# Autodesk Inventor assembly: Сборка1
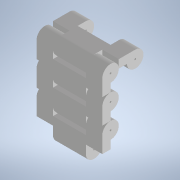
[picture p0: Inventor's stored thumbnail of the model, 180x180]
Saved by Autodesk Inventor 2020.1 (Build 241239000, 239)
## iProperties
Created: 2021-09-27
Part Number: Сборка1
Document SubType Name: Assembly
Designer: User
Author: User
## Documents named in this file (2)
- D:\GitHub\TANK\3D-TANK\Сборка1.iam
- D:\GitHub\TANK\3D-TANK\фаланга гусеницы.ipt
## Components (4 placed, 1 different names)
1. фаланга гусеницы:1 — С поворотом:1
2. фаланга гусеницы:2 — Жесткий:1, Жесткий:2
3. фаланга гусеницы:3 — С поворотом:1, Жесткий:1
4. фаланга гусеницы:5 — Жесткий:2
## Relationships (3: WeldJoint 2, RevoluteJoint 1)
- С поворотом:1 [RevoluteJoint]: фаланга гусеницы:1 ↔ фаланга гусеницы:3
- Жесткий:1 [WeldJoint]: фаланга гусеницы:2 ↔ фаланга гусеницы:3
- Жесткий:2 [WeldJoint]: фаланга гусеницы:2 ↔ фаланга гусеницы:5
